# Autodesk Inventor assembly: mat-lidar
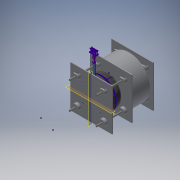
[picture p0: Inventor's stored thumbnail of the model, 180x180]
Saved by Autodesk Inventor 2019 (Build 230136000, 136)
## iProperties
Created: 2019-04-01
Part Number: mat-lidar
Document SubType Name: Assembly
Designer: franc
Author: franc
## Documents named in this file (6)
- C:\Users\franc\Desktop\EsialRobotik\Mecanique\2019\robot\mat-lidar.iam
- C:\Users\franc\Desktop\EsialRobotik\Mecanique\composants\RPlidar-A2M4\RPLIDAR A2.iam
- C:\Users\franc\Desktop\EsialRobotik\Mecanique\composants\Balises\support-balise.ipt
- C:\Users\franc\Desktop\EsialRobotik\Mecanique\composants\Balises\support-lidar.ipt
- C:\Users\franc\Desktop\EsialRobotik\Mecanique\composants\Balises\tige-filletee.ipt
- C:\Users\franc\Desktop\EsialRobotik\Mecanique\composants\Balises\cylindre-mat.ipt
## Components (9 placed, 5 different names)
1. RPLIDAR A2:1 [sub-assembly]
2. support-balise:1
3. support-lidar:1
4. tige-filletee:1
5. tige-filletee:2
6. tige-filletee:3
7. tige-filletee:4
8. support-balise:2
9. cylindre-mat:1
## Relationships (19: Mate 13, Flush 4, Tangent 2)
- [Mate]: RPLIDAR A2:1 ↔ support-lidar:1
- [Mate]: RPLIDAR A2:1 ↔ support-lidar:1
- [Mate]: RPLIDAR A2:1 ↔ support-lidar:1
- [Mate]: support-lidar:1 ↔ tige-filletee:4
- [Mate]: support-lidar:1 ↔ tige-filletee:3
- [Mate]: support-lidar:1 ↔ tige-filletee:2
- [Mate]: support-lidar:1 ↔ tige-filletee:1
- [Mate] (45 mm): support-balise:1 ↔ support-lidar:1
- [Mate]: support-balise:1 ↔ tige-filletee:1
- [Mate]: support-balise:1 ↔ tige-filletee:3
- [Flush]: tige-filletee:2 ↔ support-balise:2
- [Mate]: tige-filletee:2 ↔ support-balise:2
- [Mate]: tige-filletee:4 ↔ support-balise:2
- [Flush]: tige-filletee:4 ↔ support-balise:2
- [Flush]: tige-filletee:1 ↔ support-balise:2
- [Flush]: tige-filletee:3 ↔ support-balise:2
- [Mate]: support-balise:1 ↔ cylindre-mat:1
- [Tangent]: support-balise:1 ↔ cylindre-mat:1
- [Tangent]: support-balise:1 ↔ cylindre-mat:1
